# Autodesk Inventor assembly: socket
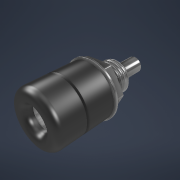
[picture p0: Inventor's stored thumbnail of the model, 180x180]
Saved by Autodesk Inventor 2022.1 (Build 261234020, 234B)
## iProperties
Created: 2021-12-02
Part Number: socket
Document SubType Name: Assembly
Designer: PaulT
Author: PaulT
## Documents named in this file (6)
- C:\Users\PaulT\OneDrive\PowerCpply\Conception\CAO\Banana socket\socket.iam
- C:\Users\PaulT\OneDrive\PowerCpply\Conception\CAO\Banana socket\screw.ipt
- C:\Users\PaulT\OneDrive\PowerCpply\Conception\CAO\Banana socket\cap_top.ipt
- C:\Users\PaulT\OneDrive\PowerCpply\Conception\CAO\Banana socket\cap_bot.ipt
- C:\Users\PaulT\OneDrive\PowerCpply\Conception\CAO\Banana socket\rondelle.ipt
- C:\Users\PaulT\OneDrive\PowerCpply\Conception\CAO\Banana socket\ecrou.ipt
## Components (5 placed, 5 different names)
1. screw:1 — Mate:2, Mate:4, Mate:5, Mate:10, Mate:11
2. cap_top:1 — Mate:10, Mate:11, Mate:12
3. cap_bot:1 — Mate:2, Mate:8, Mate:12
4. rondelle:1 — Mate:4, Mate:8, Mate:9
5. ecrou:1 — Mate:5, Mate:9
## Relationships (8: Mate 8)
- Mate:2: screw:1 ↔ cap_bot:1
- Mate:4: screw:1 ↔ rondelle:1
- Mate:5: screw:1 ↔ ecrou:1
- Mate:8: cap_bot:1 ↔ rondelle:1
- Mate:9: rondelle:1 ↔ ecrou:1
- Mate:10: screw:1 ↔ cap_top:1
- Mate:11: screw:1 ↔ cap_top:1
- Mate:12: cap_top:1 ↔ cap_bot:1
